# Autodesk Inventor assembly: lockingMechanismV03
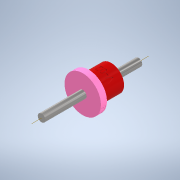
[picture p0: Inventor's stored thumbnail of the model, 180x180]
Saved by Autodesk Inventor 2021.1 (Build 251245010, 245A)
## iProperties
Created: 2020-08-16
Part Number: lockingMechanismV03
Document SubType Name: Assembly
Designer: robst
Author: robst
## Documents named in this file (6)
- C:\git\CAD-Development\robSteele\ShapeWays\TelescopeProjects\TelescopeMount\BobSteeleLockingMechanism\lockingMechanismV03.iam
- C:\git\CAD-Development\robSteele\ShapeWays\TelescopeProjects\TelescopeMount\BobSteeleLockingMechanism\5_8_inSteelRod.ipt
- C:\git\CAD-Development\robSteele\ShapeWays\TelescopeProjects\TelescopeMount\BobSteeleLockingMechanism\brake.ipt
- C:\git\CAD-Development\robSteele\ShapeWays\TelescopeProjects\TelescopeMount\BobSteeleLockingMechanism\brakeHandle.ipt
- C:\git\CAD-Development\robSteele\ShapeWays\TelescopeProjects\TelescopeMount\BobSteeleLockingMechanism\brakeLockSpacer.ipt
- C:\git\CAD-Development\robSteele\ShapeWays\TelescopeProjects\TelescopeMount\BobSteeleLockingMechanism\brakeStopAndOuterHousing.ipt
## Components (7 placed, 5 different names)
1. 5_8_inSteelRod:1 — Insert:5
2. brakeStopAndOuterHousing:1 — Insert:5, Insert:7
3. brakeHandle:1 — Insert:9
4. brakeLockSpacer:1 — Insert:7, Insert:8, Insert:9
5. brake:1 — Insert:8
6. brake:2
7. brake:3
## Component patterns: (3 elements, first: brake:1)
## Relationships (4: Insert 4)
- Insert:5 (-57.15 mm): 5_8_inSteelRod:1 ↔ brakeStopAndOuterHousing:1
- Insert:7: brakeStopAndOuterHousing:1 ↔ brakeLockSpacer:1
- Insert:8: brakeLockSpacer:1 ↔ brake:1
- Insert:9: brakeHandle:1 ↔ brakeLockSpacer:1
